# Autodesk Inventor assembly: втулка+подшипники нужная сборка_MIR_MIR
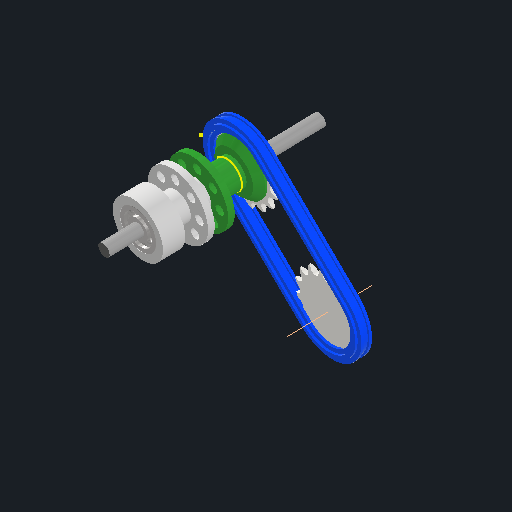
[picture p0: Inventor's stored thumbnail of the model, 512x512]
Saved by Autodesk Inventor 2025 (Build 290162000, 162)
## iProperties
Created: 2024-09-18
Part Number: втулка+подшипники нужная сборка_MIR_MIR
Document SubType Name: Assembly
Designer: GameHD
Author: Phantom
Sending System: Autodesk Inventor 2025
Preprocessor: ST-DEVELOPER v20
## Documents named in this file (5)
- C:\Users\GameHD\Downloads\Telegram Desktop\втулка+подшипники нужная сборка\втулка+подшипники нужная сборка_MIR_MIR.iam
- C:\Users\GameHD\Downloads\Telegram Desktop\втулка+подшипники нужная сборка\BS 290 SKF - SKF 626-RZ_MIR_MIR.ipt
- C:\Users\GameHD\Downloads\Telegram Desktop\втулка+подшипники нужная сборка\Деталь_64_MIR_MIR.ipt
- C:\Users\GameHD\Downloads\Telegram Desktop\втулка+подшипники нужная сборка\звезда и втулка_MIR_MIR.iam
- C:\Users\GameHD\Downloads\Telegram Desktop\втулка+подшипники нужная сборка\втулка для подш 2 часть_MIR_MIR.ipt
## Components (5 placed, 4 different names)
1. BS 290 SKF - SKF 626-RZ_MIR_MIR:1 — Совмещение:1, Совмещение:4
2. BS 290 SKF - SKF 626-RZ_MIR_MIR:2 — Совмещение:6, Совмещение:7
3. Деталь_64_MIR_MIR:1 — Совмещение:1, Совмещение:6, Совмещение:2, Совмещение:5, Совмещение:8
4. звезда и втулка_MIR_MIR:1 [sub-assembly] — Совмещение:2, Совмещение:7, Совмещение:3
5. втулка для подш 2 часть_MIR_MIR:1 — Совмещение:3, Совмещение:4, Совмещение:5, Совмещение:8
## Relationships (8: Mate 8)
- Совмещение:1 [Mate]: BS 290 SKF - SKF 626-RZ_MIR_MIR:1 ↔ Деталь_64_MIR_MIR:1
- Совмещение:6 [Mate]: BS 290 SKF - SKF 626-RZ_MIR_MIR:2 ↔ Деталь_64_MIR_MIR:1
- Совмещение:2 [Mate]: Деталь_64_MIR_MIR:1 ↔ звезда и втулка_MIR_MIR:1
- Совмещение:7 [Mate]: BS 290 SKF - SKF 626-RZ_MIR_MIR:2 ↔ звезда и втулка_MIR_MIR:1
- Совмещение:3 [Mate]: звезда и втулка_MIR_MIR:1 ↔ втулка для подш 2 часть_MIR_MIR:1
- Совмещение:4 [Mate]: BS 290 SKF - SKF 626-RZ_MIR_MIR:1 ↔ втулка для подш 2 часть_MIR_MIR:1
- Совмещение:5 [Mate]: Деталь_64_MIR_MIR:1 ↔ втулка для подш 2 часть_MIR_MIR:1
- Совмещение:8 [Mate] (15.245 mm): Деталь_64_MIR_MIR:1 ↔ втулка для подш 2 часть_MIR_MIR:1
